# Autodesk Inventor assembly: Gameboard
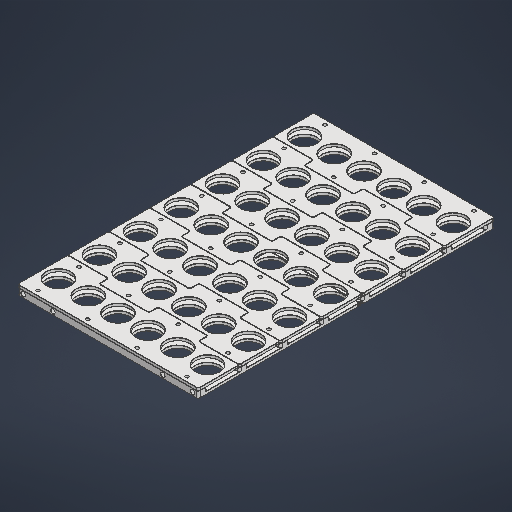
[picture p0: Inventor's stored thumbnail of the model, 512x512]
Saved by Autodesk Inventor 2025 (Build 290162010, 162A)
## iProperties
Created: 2025-12-04
Part Number: Gameboard
Document SubType Name: Assembly
Designer: FizzyApple12
Author: FizzyApple12
## Documents named in this file (4)
- C:\Users\FizzyApple12\Desktop\connect-4-robot\mcad\Gameboard\Gameboard.iam
- C:\Users\FizzyApple12\Desktop\connect-4-robot\mcad\Gameboard\Chute-Half.ipt
- C:\Users\FizzyApple12\Desktop\connect-4-robot\mcad\Gameboard\Backer.ipt
- C:\Users\FizzyApple12\Desktop\connect-4-robot\mcad\Gameboard\Backer-End.ipt
## Components (9 placed, 3 different names)
1. Chute-Half:1 — Flush:1, Flush:2, Mate:7, Mate:10, Mate:11, Mate:15, Mate:16, Mate:17, Mate:18, Mate:26, Mate:27, Mate:28
2. Chute-Half:2 — Flush:1, Flush:2, Mate:5, Mate:6, Mate:8, Mate:9, Mate:19, Mate:20, Mate:21, Mate:22, Mate:23, Mate:24, Mate:25
3. Backer:2 — Mate:5, Mate:6, Mate:7
4. Backer:3 — Mate:8, Mate:21, Mate:22
5. Backer:4 — Mate:9, Mate:19, Mate:20
6. Backer:5 — Mate:10, Mate:17, Mate:18
7. Backer:6 — Mate:11, Mate:15, Mate:16
8. Backer-End:1 — Mate:26, Mate:27, Mate:28
9. Backer-End:2 — Mate:23, Mate:24, Mate:25
## Relationships (23: Mate 21, Flush 2)
- Flush:1: Chute-Half:1 ↔ Chute-Half:2
- Flush:2: Chute-Half:1 ↔ Chute-Half:2
- Mate:5: Chute-Half:2 ↔ Backer:2
- Mate:6: Chute-Half:2 ↔ Backer:2
- Mate:7: Chute-Half:1 ↔ Backer:2
- Mate:8: Chute-Half:2 ↔ Backer:3
- Mate:9: Chute-Half:2 ↔ Backer:4
- Mate:10: Chute-Half:1 ↔ Backer:5
- Mate:11: Chute-Half:1 ↔ Backer:6
- Mate:15: Chute-Half:1 ↔ Backer:6
- Mate:16: Chute-Half:1 ↔ Backer:6
- Mate:17: Chute-Half:1 ↔ Backer:5
- Mate:18: Chute-Half:1 ↔ Backer:5
- Mate:19: Chute-Half:2 ↔ Backer:4
- Mate:20: Chute-Half:2 ↔ Backer:4
- Mate:21: Chute-Half:2 ↔ Backer:3
- Mate:22: Chute-Half:2 ↔ Backer:3
- Mate:23: Chute-Half:2 ↔ Backer-End:2
- Mate:24: Chute-Half:2 ↔ Backer-End:2
- Mate:25: Chute-Half:2 ↔ Backer-End:2
- Mate:26: Chute-Half:1 ↔ Backer-End:1
- Mate:27: Chute-Half:1 ↔ Backer-End:1
- Mate:28: Chute-Half:1 ↔ Backer-End:1
